# Autodesk Inventor assembly: Assembly23-02-2022
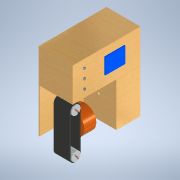
[picture p0: Inventor's stored thumbnail of the model, 180x180]
Saved by Autodesk Inventor 2022.2 (Build 262287000, 287)
## iProperties
Created: 2022-02-23
Part Number: Assembly23-02-2022
Document SubType Name: Assembly
Designer: PRASHANTH
Author: PRASHANTH
## Documents named in this file (9)
- E:\BME\Autodesk Sample\Assembly23-02-2022.iam
- E:\BME\Autodesk Sample\Assembly of Conveyor Belt.iam
- E:\BME\Autodesk Sample\Body Skeleton.ipt
- E:\BME\Autodesk Sample\Side Part.ipt
- E:\BME\Autodesk Sample\Square.ipt
- E:\BME\Autodesk Sample\Aurdino.ipt
- E:\BME\Autodesk Sample\Buttons.ipt
- E:\BME\Autodesk Sample\Compartment Division.ipt
- E:\BME\Autodesk Sample\box.ipt
## Components (13 placed, 8 different names)
1. Assembly of Conveyor Belt:1 [sub-assembly] — Flush:5, Mate:14
2. Body Skeleton:1 — Mate:1, Flush:1, Flush:2, Mate:2, Flush:3, Flush:4, Flush:5, Mate:3, Flush:7, Mate:8, Mate:10, Mate:12
3. Side Part:1 — Mate:2, Flush:3, Flush:4, Flush:6, Mate:9, Mate:11, Mate:13
4. Side Part:2 — Mate:1, Flush:1, Flush:2, Mate:4, Flush:8, Flush:9, Mate:5, Mate:6, Mate:7
5. Square:1 — Flush:6, Mate:3, Flush:7
6. Aurdino:1 — Mate:4, Flush:8, Flush:9
7. Buttons:1 — Mate:7, Flush:10, Flush:11
8. Buttons:2 — Mate:6, Flush:10
9. Buttons:3 — Mate:5, Flush:11
10. Compartment Division:1 — Mate:8, Mate:9
11. Compartment Division:2 — Mate:12, Mate:13
12. Compartment Division:3 — Mate:10, Mate:11
13. box:1 — Mate:14
## Relationships (25: Mate 14, Flush 11)
- Mate:1: Body Skeleton:1 ↔ Side Part:2
- Flush:1: Body Skeleton:1 ↔ Side Part:2
- Flush:2: Body Skeleton:1 ↔ Side Part:2
- Mate:2: Body Skeleton:1 ↔ Side Part:1
- Flush:3: Body Skeleton:1 ↔ Side Part:1
- Flush:4: Body Skeleton:1 ↔ Side Part:1
- Flush:5 (-200 mm): Assembly of Conveyor Belt:1 ↔ Body Skeleton:1
- Flush:6: Side Part:1 ↔ Square:1
- Mate:3: Body Skeleton:1 ↔ Square:1
- Flush:7: Body Skeleton:1 ↔ Square:1
- Mate:4: Side Part:2 ↔ Aurdino:1
- Flush:8 (55 mm): Side Part:2 ↔ Aurdino:1
- Flush:9 (40 mm): Side Part:2 ↔ Aurdino:1
- Mate:5: Side Part:2 ↔ Buttons:3
- Mate:6: Side Part:2 ↔ Buttons:2
- Mate:7: Side Part:2 ↔ Buttons:1
- Flush:10: Buttons:1 ↔ Buttons:2
- Flush:11: Buttons:1 ↔ Buttons:3
- Mate:8: Body Skeleton:1 ↔ Compartment Division:1
- Mate:9: Side Part:1 ↔ Compartment Division:1
- Mate:10: Body Skeleton:1 ↔ Compartment Division:3
- Mate:11: Side Part:1 ↔ Compartment Division:3
- Mate:12: Body Skeleton:1 ↔ Compartment Division:2
- Mate:13: Side Part:1 ↔ Compartment Division:2
- Mate:14: Assembly of Conveyor Belt:1 ↔ box:1
